# Autodesk Inventor assembly: main_led_strip
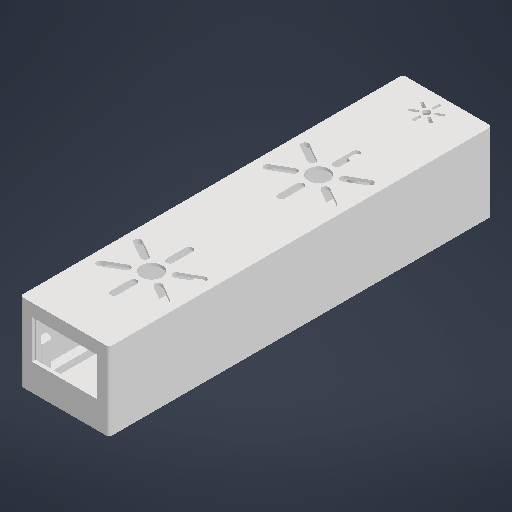
[picture p0: Inventor's stored thumbnail of the model, 512x512]
Saved by Autodesk Inventor 2027 (Build 310192060, 192F)
## iProperties
Created: 2026-08-21
Part Number: main_led_strip
Document SubType Name: Assembly
Designer: User
Author: User
## Documents named in this file (3)
- G:\Github\SmartRoom\Hardware\SmartRoom_Led_Strip\main_led_strip.iam
- G:\Github\SmartRoom\Hardware\SmartRoom_Led_Strip\Parts\base.ipt
- G:\Github\SmartRoom\Hardware\SmartRoom_Led_Strip\Parts\top.ipt
## Components (2 placed, 2 different names)
1. base:1 — Obrotowe:1, Obrotowe:2
2. top:1 — Obrotowe:1, Obrotowe:2
## Relationships (2: RevoluteJoint 2)
- Obrotowe:1 [RevoluteJoint]: base:1 ↔ top:1
- Obrotowe:2 [RevoluteJoint]: base:1 ↔ top:1
